# Autodesk Inventor assembly: +XPanel
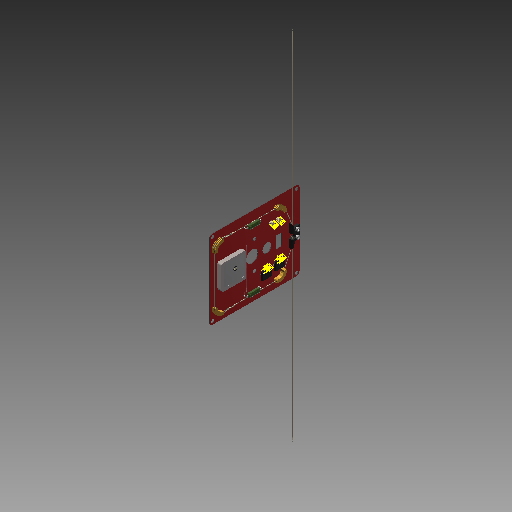
[picture p0: Inventor's stored thumbnail of the model, 512x512]
Saved by Autodesk Inventor 2018 (Build 220112000, 112)
## iProperties
Created: 2018-10-25
Part Number: +XPanel
Document SubType Name: Assembly
Designer: Bradley
Author: Bradley
## Documents named in this file (14)
- C:\Users\Bradley\Documents\GitHub\CougSat1-Hardware\CougSat1-RadioBoard\CADModel\Native\+XPanel.iam
- C:\Users\Bradley\Documents\GitHub\CougSat1-Hardware\CougSat1-RadioBoard\CADModel\Native\+XPanel_PCB.ipt
- C:\Users\Bradley\Documents\GitHub\CougSat1-Hardware\CougSat1-RadioBoard\CADModel\Native\+XPanel_AntennaPost.ipt
- C:\Users\Bradley\Documents\GitHub\CougSat1-Hardware\CougSat1-RadioBoard\CADModel\Native\+XPanel_AntennaMount.ipt
- C:\Users\Bradley\Documents\GitHub\CougSat1-Hardware\CougSat1-RadioBoard\CADModel\Native\+XPanel_AntennaStored+Y.ipt
- C:\Users\Bradley\Documents\GitHub\CougSat1-Hardware\CougSat1-RadioBoard\CADModel\Native\+XPanel_AntennaStored-Y.ipt
- C:\Users\Bradley\Documents\GitHub\CougSat1-Hardware\CougSat1-RadioBoard\CADModel\Native\+XPanel_AntennaString.ipt
- C:\Users\Bradley\Documents\GitHub\CougSat1-Hardware\CougSat1-RadioBoard\CADModel\Native\+XPanel_AntennaDeployed.ipt
- C:\Users\Bradley\Documents\GitHub\Resources\SupplierDocuments\04 - Connectors SMT\04-0001\04-0001.iam
- C:\Users\Bradley\Documents\GitHub\Resources\SupplierDocuments\25 - Resistor THT\25-15.0\25-15.0.ipt
- C:\Users\Bradley\Documents\GitHub\Resources\SupplierDocuments\04 - Connectors SMT\04-0008\04-0008.iam
- C:\Users\Bradley\Documents\GitHub\Resources\SupplierDocuments\65 - RF\65-0010\65-0010.ipt
- C:\Users\Bradley\Documents\GitHub\Resources\SupplierDocuments\48 - Hardware\48-0240\48-0240.ipt
- C:\Users\Bradley\Documents\GitHub\Resources\SupplierDocuments\48 - Hardware\48-0074\48-0074.ipt
## Components (23 placed, 13 different names)
1. 04-0001:1 [sub-assembly] — Mate:5, Flush:3, Mate:6
2. 04-0001:2 [sub-assembly] — Mate:28, Mate:29, Flush:7
3. 04-0008:1 [sub-assembly] — Angle:1
4. 04-0008:2 [sub-assembly] — Angle:2
5. 25-15.0:1 — Insert:17, Insert:18, Mate:19, Mate:23
6. 25-15.0:2 — Insert:19, Insert:20, Mate:20, Mate:22
7. 48-0240:1 — Insert:13
8. 48-0240:2 — Insert:14
9. 48-0074:1 — Insert:9
10. 48-0074:2 — Insert:10
11. 65-0010:1 — Insert:1, Flush:1
12. +XPanel_AntennaDeployed:1 — Mate:24, Mate:25
13. +XPanel_AntennaDeployed:2 — Mate:26, Mate:27
14. +XPanel_AntennaMount:1 — Insert:11, Insert:12, Insert:13, Insert:14, Mate:25, Mate:27
15. +XPanel_AntennaPost:1 — Insert:4, Mate:9
16. +XPanel_AntennaPost:2 — Insert:8, Mate:10
17. +XPanel_AntennaPost:3 — Insert:7, Mate:11, Mate:13, Mate:17
18. +XPanel_AntennaPost:4 — Insert:6, Mate:12, Mate:15, Mate:16
19. +XPanel_AntennaStored+Y:1 — Mate:13, Mate:14, Mate:15
20. +XPanel_AntennaStored-Y:1 — Mate:16, Mate:17, Mate:18
21. +XPanel_AntennaString:1 — Mate:19, Mate:20, Flush:6
22. +XPanel_AntennaString:2 — Mate:21, Mate:22, Mate:23
23. +XPanel_PCB:1 — Insert:1, Insert:4, Insert:6, Insert:7, Insert:8, Insert:9, Insert:10, Insert:11, Insert:12, Mate:5, Mate:9, Mate:10, Mate:11, Mate:12, Mate:14, Mate:18, Insert:17, Insert:18, Insert:19, Insert:20, Mate:24, Mate:26, Mate:28
## Relationships (44: Mate 23, Insert 15, Flush 4, Angle 2)
- Insert:1: 65-0010:1 ↔ +XPanel_PCB:1
- Flush:1: 65-0010:1
- Insert:4: +XPanel_AntennaPost:1 ↔ +XPanel_PCB:1
- Insert:6: +XPanel_AntennaPost:4 ↔ +XPanel_PCB:1
- Insert:7: +XPanel_AntennaPost:3 ↔ +XPanel_PCB:1
- Insert:8: +XPanel_AntennaPost:2 ↔ +XPanel_PCB:1
- Insert:9: 48-0074:1 ↔ +XPanel_PCB:1
- Insert:10: 48-0074:2 ↔ +XPanel_PCB:1
- Insert:11: +XPanel_AntennaMount:1 ↔ +XPanel_PCB:1
- Insert:12: +XPanel_AntennaMount:1 ↔ +XPanel_PCB:1
- Insert:13: 48-0240:1 ↔ +XPanel_AntennaMount:1
- Insert:14: 48-0240:2 ↔ +XPanel_AntennaMount:1
- Mate:5: 04-0001:1 ↔ +XPanel_PCB:1
- Flush:3 (23 mm): 04-0001:1
- Mate:6 (-24 mm): 04-0001:1
- Angle:1 (30 deg): 04-0008:1
- Angle:2 (30 deg): 04-0008:2
- Mate:9: +XPanel_AntennaPost:1 ↔ +XPanel_PCB:1
- Mate:10: +XPanel_AntennaPost:2 ↔ +XPanel_PCB:1
- Mate:11: +XPanel_AntennaPost:3 ↔ +XPanel_PCB:1
- Mate:12: +XPanel_AntennaPost:4 ↔ +XPanel_PCB:1
- Mate:13: +XPanel_AntennaPost:3 ↔ +XPanel_AntennaStored+Y:1
- Mate:14 (2.5 mm): +XPanel_AntennaStored+Y:1 ↔ +XPanel_PCB:1
- Mate:15: +XPanel_AntennaPost:4 ↔ +XPanel_AntennaStored+Y:1
- Mate:16: +XPanel_AntennaPost:4 ↔ +XPanel_AntennaStored-Y:1
- Mate:17: +XPanel_AntennaPost:3 ↔ +XPanel_AntennaStored-Y:1
- Mate:18 (1 mm): +XPanel_AntennaStored-Y:1 ↔ +XPanel_PCB:1
- Insert:17 (-1 mm): 25-15.0:1 ↔ +XPanel_PCB:1
- Insert:18 (-1 mm): 25-15.0:1 ↔ +XPanel_PCB:1
- Insert:19 (-1 mm): 25-15.0:2 ↔ +XPanel_PCB:1
- Insert:20 (-1 mm): 25-15.0:2 ↔ +XPanel_PCB:1
- Mate:19: 25-15.0:1 ↔ +XPanel_AntennaString:1
- Mate:20: 25-15.0:2 ↔ +XPanel_AntennaString:1
- Flush:6 (2.8 mm): +XPanel_AntennaString:1
- Mate:21 (1.3 mm): +XPanel_AntennaString:2
- Mate:22: 25-15.0:2 ↔ +XPanel_AntennaString:2
- Mate:23: 25-15.0:1 ↔ +XPanel_AntennaString:2
- Mate:24: +XPanel_AntennaDeployed:1 ↔ +XPanel_PCB:1
- Mate:25: +XPanel_AntennaDeployed:1 ↔ +XPanel_AntennaMount:1
- Mate:26: +XPanel_AntennaDeployed:2 ↔ +XPanel_PCB:1
- Mate:27: +XPanel_AntennaDeployed:2 ↔ +XPanel_AntennaMount:1
- Mate:28: 04-0001:2 ↔ +XPanel_PCB:1
- Mate:29 (-11 mm): 04-0001:2
- Flush:7 (25 mm): 04-0001:2
